# Autodesk Inventor assembly: ECDL
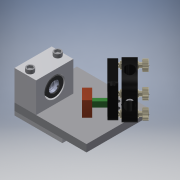
[picture p0: Inventor's stored thumbnail of the model, 180x180]
Saved by Autodesk Inventor 2019.4 (Build 234330000, 330)
## iProperties
Created: 2018-03-23
Part Number: ECDL
Document SubType Name: Assembly
Designer: Hogar
Author: Hogar
## Documents named in this file (11)
- E:\pixki\OCR\Designs\lasers\ECDL OCR\ECDL.iam
- E:\pixki\OCR\Designs\lasers\ECDL OCR\Base.ipt
- E:\pixki\OCR\Designs\lasers\ECDL OCR\Peltier.ipt
- E:\pixki\OCR\Designs\lasers\ECDL OCR\Colimador inferior.ipt
- E:\pixki\OCR\Designs\lasers\ECDL OCR\Colimador superior.ipt
- E:\pixki\OCR\Designs\lasers\ECDL OCR\LT110P-B-Solidworks.ipt
- E:\pixki\OCR\Designs\lasers\ECDL OCR\Newfocus_9882.ipt
- E:\pixki\OCR\Designs\lasers\ECDL OCR\M4 sujecion.ipt
- E:\pixki\OCR\Designs\lasers\ECDL OCR\PZT.ipt
- E:\pixki\OCR\Designs\lasers\ECDL OCR\GH.ipt
- E:\pixki\OCR\Designs\lasers\ECDL OCR\M4 union.ipt
## Components (11 placed, 10 different names)
1. Base:1 — Mate:1, Mate:2, Mate:3, Mate:4, Flush:1, Flush:2, Mate:5, Mate:6, Mate:7, Mate:12, Angle:1, Mate:13, Mate:14, Flush:3, Angle:2, Angle:3
2. Peltier:1 — Mate:4, Flush:1, Flush:2
3. Colimador inferior:1 — Mate:5, Mate:6, Mate:7, Mate:8, Mate:9, Mate:10, Mate:11
4. Colimador superior:1 — Mate:8, Mate:9, Mate:10, Mate:20, Mate:21, Mate:22, Mate:23
5. LT110P-B-Solidworks:1 — Mate:11
6. Newfocus_9882:1 — Mate:12, Angle:1, Mate:13, Mate:15, Flush:4, Flush:5
7. M4 sujecion:1 — Mate:14, Mate:15
8. PZT:1 — Mate:18, Angle:2, Flush:5, Mate:19, Flush:6, Flush:7
9. GH:1 — Mate:19, Angle:3, Flush:6, Flush:7
10. M4 union:1 — Mate:20, Mate:22
11. M4 union:2 — Mate:21, Mate:23
## Relationships (33: Mate 23, Flush 7, Angle 3)
- Mate:1: Base:1
- Mate:2: Base:1
- Mate:3 (-52 mm): Base:1
- Mate:4: Base:1 ↔ Peltier:1
- Flush:1: Base:1 ↔ Peltier:1
- Flush:2: Base:1 ↔ Peltier:1
- Mate:5: Base:1 ↔ Colimador inferior:1
- Mate:6: Base:1 ↔ Colimador inferior:1
- Mate:7: Base:1 ↔ Colimador inferior:1
- Mate:8: Colimador inferior:1 ↔ Colimador superior:1
- Mate:9: Colimador inferior:1 ↔ Colimador superior:1
- Mate:10: Colimador inferior:1 ↔ Colimador superior:1
- Mate:11: Colimador inferior:1 ↔ LT110P-B-Solidworks:1
- Mate:12: Base:1 ↔ Newfocus_9882:1
- Angle:1 (45 deg): Base:1 ↔ Newfocus_9882:1
- Mate:13: Base:1 ↔ Newfocus_9882:1
- Mate:14: Base:1 ↔ M4 sujecion:1
- Mate:15: Newfocus_9882:1 ↔ M4 sujecion:1
- Flush:3 (12.5 mm): Base:1
- Flush:4: Newfocus_9882:1
- Mate:16
- Mate:17
- Mate:18: PZT:1
- Angle:2 (0 deg): Base:1 ↔ PZT:1
- Flush:5 (-3.247 mm): Newfocus_9882:1 ↔ PZT:1
- Mate:19: PZT:1 ↔ GH:1
- Angle:3 (0 deg): Base:1 ↔ GH:1
- Flush:6 (4.6 mm): PZT:1 ↔ GH:1
- Flush:7 (4.1 mm): PZT:1 ↔ GH:1
- Mate:20: Colimador superior:1 ↔ M4 union:1
- Mate:21: Colimador superior:1 ↔ M4 union:2
- Mate:22: Colimador superior:1 ↔ M4 union:1
- Mate:23: Colimador superior:1 ↔ M4 union:2
